# Autodesk Inventor assembly: MECANISMO DE COMPACTADO
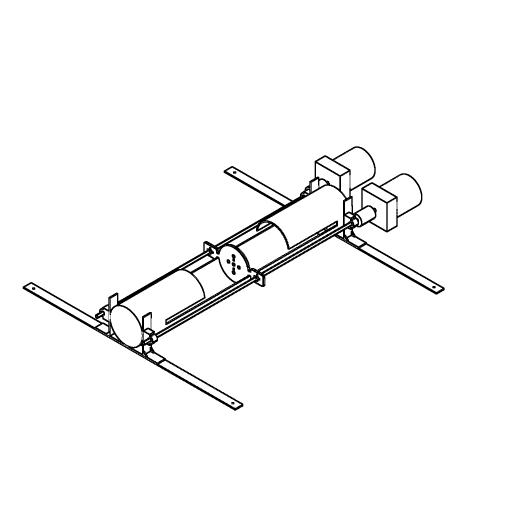
[picture p0: Inventor's stored thumbnail of the model, 512x512]
Saved by Autodesk Inventor 2024 (Build 280153000, 153)
## iProperties
Created: 2024-05-26
Part Number: MECANISMO DE COMPACTADO
Document SubType Name: Assembly
Designer: Jhuliams
Author: Jhuliams
## Documents named in this file (10)
- C:\Users\Jhuliams\Documents\GitHub\RECICLADOR_MODELO_3D\MECANISMO DE COMPACTADO\MECANISMO DE COMPACTADO.iam
- C:\Users\Jhuliams\Documents\GitHub\RECICLADOR_MODELO_3D\MECANISMO DE COMPACTADO\GUIA_DE_OBJETO.ipt
- C:\Users\Jhuliams\Documents\GitHub\RECICLADOR_MODELO_3D\MECANISMO DE COMPACTADO\TAPA QUE DESPLAZA CON TORNILLOS.ipt
- C:\Users\Jhuliams\Documents\GitHub\RECICLADOR_MODELO_3D\MECANISMO DE COMPACTADO\TUERCA DE HUSILLO.ipt
- C:\Users\Jhuliams\Documents\GitHub\RECICLADOR_MODELO_3D\MECANISMO DE COMPACTADO\TORNILLO DEPOTENCIA.ipt
- C:\Users\Jhuliams\Documents\GitHub\RECICLADOR_MODELO_3D\MECANISMO DE COMPACTADO\SOPORTE DE GUIA.ipt
- C:\Users\Jhuliams\Documents\GitHub\RECICLADOR_MODELO_3D\MECANISMO DE COMPACTADO\ACOPLE HELICOIDAL.ipt
- C:\Users\Jhuliams\Documents\GitHub\RECICLADOR_MODELO_3D\MECANISMO DE COMPACTADO\MOTOR DC.ipt
- C:\Users\Jhuliams\Documents\GitHub\RECICLADOR_MODELO_3D\MECANISMO DE COMPACTADO\RODAMIENTO DE TORNILLO.ipt
- C:\Users\Jhuliams\Documents\GitHub\RECICLADOR_MODELO_3D\MECANISMO DE COMPACTADO\PLETINA PARA GUIA CILINDRICA.ipt
## Components (18 placed, 9 different names)
1. GUIA_DE_OBJETO:1 — Mate:54, Tangent:1, Tangent:2, Flush:17, Tangent:3, Tangent:4, Mate:60, Mate:61
2. ACOPLE HELICOIDAL:1 — Mate:36, Mate:38, Mate:42, Mate:43
3. ACOPLE HELICOIDAL:2 — Mate:35, Mate:37, Mate:41, Mate:44
4. RODAMIENTO DE TORNILLO:1 — Flush:12, Flush:19, Mate:58
5. RODAMIENTO DE TORNILLO:2 — Flush:11, Flush:20, Mate:59, Flush:23
6. PLETINA PARA GUIA CILINDRICA:1 — Mate:56, Flush:16, Flush:24
7. PLETINA PARA GUIA CILINDRICA:2 — Mate:57, Flush:18
8. MOTOR DC:1 — Mate:35, Mate:37
9. MOTOR DC:2 — Mate:36, Mate:38
10. TORNILLO DEPOTENCIA:1 — Flush:11, Mate:42, Mate:43, Mate:47, Mate:49, Mate:59
11. TORNILLO DEPOTENCIA:2 — Flush:12, Mate:41, Mate:44, Mate:45, Mate:50, Mate:58
12. RODAMIENTO DE TORNILLO:3 — Mate:45, Flush:21
13. RODAMIENTO DE TORNILLO:4 — Mate:47, Flush:22
14. TUERCA DE HUSILLO:1 — Mate:49, Flush:15, Mate:55
15. TUERCA DE HUSILLO:2 — Mate:50, Flush:15, Mate:52, Mate:53
16. TAPA QUE DESPLAZA CON TORNILLOS:1 — Mate:52, Mate:53, Mate:54, Mate:55, Mate:60, Mate:61
17. SOPORTE DE GUIA:1 — Tangent:1, Mate:56, Tangent:2, Flush:16, Flush:17, Flush:19, Flush:20, Flush:23, Flush:24
18. SOPORTE DE GUIA:2 — Tangent:3, Tangent:4, Mate:57, Flush:18, Flush:21, Flush:22
## Relationships (38: Mate 22, Flush 12, Tangent 4)
- Mate:35: ACOPLE HELICOIDAL:2 ↔ MOTOR DC:1
- Mate:36: ACOPLE HELICOIDAL:1 ↔ MOTOR DC:2
- Mate:37 (12 mm): ACOPLE HELICOIDAL:2 ↔ MOTOR DC:1
- Mate:38 (12 mm): ACOPLE HELICOIDAL:1 ↔ MOTOR DC:2
- Flush:11 (-20 mm): RODAMIENTO DE TORNILLO:2 ↔ TORNILLO DEPOTENCIA:1
- Flush:12 (-20 mm): RODAMIENTO DE TORNILLO:1 ↔ TORNILLO DEPOTENCIA:2
- Mate:41: ACOPLE HELICOIDAL:2 ↔ TORNILLO DEPOTENCIA:2
- Mate:42: ACOPLE HELICOIDAL:1 ↔ TORNILLO DEPOTENCIA:1
- Mate:43 (-15 mm): ACOPLE HELICOIDAL:1 ↔ TORNILLO DEPOTENCIA:1
- Mate:44 (-15 mm): ACOPLE HELICOIDAL:2 ↔ TORNILLO DEPOTENCIA:2
- Mate:45: TORNILLO DEPOTENCIA:2 ↔ RODAMIENTO DE TORNILLO:3
- Mate:47: TORNILLO DEPOTENCIA:1 ↔ RODAMIENTO DE TORNILLO:4
- Mate:49: TORNILLO DEPOTENCIA:1 ↔ TUERCA DE HUSILLO:1
- Mate:50: TORNILLO DEPOTENCIA:2 ↔ TUERCA DE HUSILLO:2
- Flush:15: TUERCA DE HUSILLO:1 ↔ TUERCA DE HUSILLO:2
- Mate:52: TUERCA DE HUSILLO:2 ↔ TAPA QUE DESPLAZA CON TORNILLOS:1
- Mate:53: TUERCA DE HUSILLO:2 ↔ TAPA QUE DESPLAZA CON TORNILLOS:1
- Mate:54: GUIA_DE_OBJETO:1 ↔ TAPA QUE DESPLAZA CON TORNILLOS:1
- Mate:55: TUERCA DE HUSILLO:1 ↔ TAPA QUE DESPLAZA CON TORNILLOS:1
- Tangent:1: GUIA_DE_OBJETO:1 ↔ SOPORTE DE GUIA:1
- Mate:56: PLETINA PARA GUIA CILINDRICA:1 ↔ SOPORTE DE GUIA:1
- Tangent:2: GUIA_DE_OBJETO:1 ↔ SOPORTE DE GUIA:1
- Flush:16: PLETINA PARA GUIA CILINDRICA:1 ↔ SOPORTE DE GUIA:1
- Flush:17: GUIA_DE_OBJETO:1 ↔ SOPORTE DE GUIA:1
- Tangent:3: GUIA_DE_OBJETO:1 ↔ SOPORTE DE GUIA:2
- Tangent:4: GUIA_DE_OBJETO:1 ↔ SOPORTE DE GUIA:2
- Mate:57: PLETINA PARA GUIA CILINDRICA:2 ↔ SOPORTE DE GUIA:2
- Flush:18: PLETINA PARA GUIA CILINDRICA:2 ↔ SOPORTE DE GUIA:2
- Flush:19: RODAMIENTO DE TORNILLO:1 ↔ SOPORTE DE GUIA:1
- Flush:20: RODAMIENTO DE TORNILLO:2 ↔ SOPORTE DE GUIA:1
- Mate:58: RODAMIENTO DE TORNILLO:1 ↔ TORNILLO DEPOTENCIA:2
- Mate:59: RODAMIENTO DE TORNILLO:2 ↔ TORNILLO DEPOTENCIA:1
- Flush:21: RODAMIENTO DE TORNILLO:3 ↔ SOPORTE DE GUIA:2
- Flush:22: RODAMIENTO DE TORNILLO:4 ↔ SOPORTE DE GUIA:2
- Flush:23: RODAMIENTO DE TORNILLO:2 ↔ SOPORTE DE GUIA:1
- Flush:24 (250 mm): PLETINA PARA GUIA CILINDRICA:1 ↔ SOPORTE DE GUIA:1
- Mate:60 (1 mm): GUIA_DE_OBJETO:1 ↔ TAPA QUE DESPLAZA CON TORNILLOS:1
- Mate:61 (1 mm): GUIA_DE_OBJETO:1 ↔ TAPA QUE DESPLAZA CON TORNILLOS:1
